# Autodesk Inventor assembly: EFS Mark I
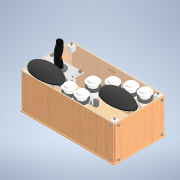
[picture p0: Inventor's stored thumbnail of the model, 180x180]
Saved by Autodesk Inventor 2022 (Build 260153000, 153)
## iProperties
Category: Gaming
Company: El Camino College
Created: 2023-03-29
Part Number: EFS Mark I
Document SubType Name: Assembly
Designer: Edgar Tejada
Project: Ergonomic Fight Stick
Mass: 952.379 g
Surface Area: 5483.02 cm^2
Volume: 844.231 cm^3
Density: 1.1281 g/cm^3
Author: Edgar Tejada
Title: Ergonomic Fight Stick
Keywords: Gaming Arcade Mame Ergonomic
## Documents named in this file (15)
- G:\Documents\Inventor HW\Ergonomic Fight Stick\Ergonomic_Fight_Stick.iam
- G:\Documents\Inventor HW\Ergonomic Fight Stick\Base_Plate.ipt
- G:\Documents\Inventor HW\Ergonomic Fight Stick\Vertical_Plate.ipt
- G:\Documents\Inventor HW\Ergonomic Fight Stick\Horizontal_Plate.ipt
- G:\Documents\Inventor HW\Ergonomic Fight Stick\Corner_M3_Mounts.ipt
- G:\Documents\Inventor HW\Ergonomic Fight Stick\AS 1420 - 1973 - M3 x 6.ipt
- G:\Documents\Inventor HW\Ergonomic Fight Stick\Top_Plate.ipt
- G:\Documents\Inventor HW\Ergonomic Fight Stick\Pushbutton - BG.iam
- G:\Documents\Inventor HW\Ergonomic Fight Stick\Sanwa JLF-TP-8YT 16Gate.iam
- G:\Documents\Inventor HW\Ergonomic Fight Stick\Makey_Makey_Circuit_Board.ipt
- C:\Users\brev\Documents\Inventor\Content Center Files\R2022\en-US\AS 1420\AS 1420 - 1973 - M3 x 10.ipt
- C:\Users\brev\Documents\Inventor\Content Center Files\R2022\en-US\BS 4183(1)\BS 4183 - M3(1).ipt
- G:\Documents\Inventor HW\Ergonomic Fight Stick\Nagasuye_Ergonomic_Controller_New_Grip.ipt
- G:\Documents\Inventor HW\Ergonomic Fight Stick\Silicone_Wrist_Support.ipt
- C:\Users\brev\Documents\Inventor\Content Center Files\R2022\en-US\SS-ISO 7093\ISO 7093 - 3 - 140 HV(2).ipt
## Components (67 placed, 14 different names)
1. Base_Plate:1 — Mate:1, Mate:2, Mate:3, Mate:4, Tangent:1, Tangent:2, Mate:5, Mate:6, Mate:7, Mate:8, Tangent:3, Tangent:4, Mate:9, Mate:10, Mate:11, Mate:12, Insert:3, Insert:6, Insert:8, Insert:9, Angle:4, Insert:32, Insert:33, Insert:34, Angle:8, Insert:35, Angle:10, Flush:1
2. Vertical_Plate:1 — Mate:1, Mate:3, Tangent:1, Insert:1, Insert:5, Angle:1, Insert:21, Insert:22
3. Vertical_Plate:2 — Mate:2, Mate:4, Tangent:2, Insert:12, Insert:13, Angle:3, Insert:19, Insert:25, Angle:5
4. Horizontal_Plate:3 — Mate:5, Mate:8, Tangent:4, Insert:7, Insert:11, Angle:2, Insert:23, Insert:24
5. Horizontal_Plate:4 — Mate:6, Mate:7, Tangent:3, Insert:10, Insert:17, Insert:18, Angle:6, Angle:9
6. AS 1420 - Metric M3 x 6:1 — Insert:1, Insert:2
7. AS 1420 - Metric M3 x 6:3 — Insert:4
8. AS 1420 - Metric M3 x 6:6 — Insert:11
9. AS 1420 - Metric M3 x 6:8 — Insert:13
10. AS 1420 - Metric M3 x 6:9 — Insert:7
11. AS 1420 - Metric M3 x 6:10 — Insert:10
12. AS 1420 - Metric M3 x 6:11 — Insert:12
13. AS 1420 - Metric M3 x 6:12 — Insert:5
14. AS 1420 - Metric M3 x 6:13 — Insert:17
15. AS 1420 - Metric M3 x 6:14 — Insert:18
16. AS 1420 - Metric M3 x 6:15 — Insert:19
17. AS 1420 - Metric M3 x 6:16 — Insert:25
18. AS 1420 - Metric M3 x 6:17 — Insert:21
19. AS 1420 - Metric M3 x 6:18 — Insert:22
20. AS 1420 - Metric M3 x 6:19 — Insert:24
21. AS 1420 - Metric M3 x 6:20 — Insert:23
22. Top_Plate:1 — Angle:4, Angle:5, Angle:6, Insert:26, Insert:27, Insert:28, Insert:29, Insert:30, Mate:13, Insert:31, Angle:7, Angle:10, Flush:1, Mate:15, Mate:16, Insert:39, Insert:40, Insert:41, Insert:42, Insert:43, Insert:44, Insert:45, Insert:46, Angle:11, Angle:12, Angle:14, Mate:19, Mate:20
23. Pushbutton - BG:1 [sub-assembly] — Insert:30
24. Pushbutton - BG:2 [sub-assembly] — Insert:29
25. Pushbutton - BG:3 [sub-assembly] — Mate:13
26. Pushbutton - BG:4 [sub-assembly] — Insert:28
27. Pushbutton - BG:5 [sub-assembly] — Insert:27
28. Pushbutton - BG:6 [sub-assembly] — Insert:26
29. Sanwa JLF-TP-8YT 16Gate:1 [sub-assembly] — Insert:31, Angle:7, Insert:51
30. AS 1420 - Metric M3 x 10:1 — Insert:32
31. AS 1420 - Metric M3 x 10:3 — Insert:34
32. AS 1420 - Metric M3 x 10:2 — Insert:33
33. Makey_Makey_Circuit_Board:1 — Angle:8, Insert:35, Angle:9, Insert:36, Insert:37, Insert:38
34. BS 4183 - Metric M3:1 — Insert:36
35. BS 4183 - Metric M3:2 — Insert:38
36. BS 4183 - Metric M3:3 — Insert:37
37. AS 1420 - Metric M3 x 6:5 — Insert:6, Insert:14
38. AS 1420 - Metric M3 x 6:7 — Insert:9, Insert:15
39. AS 1420 - Metric M3 x 6:4 — Insert:8, Insert:16
40. AS 1420 - Metric M3 x 6:2 — Insert:3
41. AS 1420 - Metric M3 x 6:21 — Insert:39, Insert:48, Insert:52
42. AS 1420 - Metric M3 x 6:22 — Insert:41, Insert:49, Insert:54
43. AS 1420 - Metric M3 x 6:23 — Insert:43
44. AS 1420 - Metric M3 x 6:24 — Insert:40, Insert:50, Insert:53
45. AS 1420 - Metric M3 x 6:25 — Insert:46
46. AS 1420 - Metric M3 x 6:26 — Insert:44
47. AS 1420 - Metric M3 x 6:27 — Insert:42, Insert:47, Insert:55
48. AS 1420 - Metric M3 x 6:28 — Insert:45
49. BS 4183 - Metric M3:4 — Insert:47
50. BS 4183 - Metric M3:5 — Insert:48
51. BS 4183 - Metric M3:6 — Insert:50
52. BS 4183 - Metric M3:7 — Insert:49
53. Nagasuye_Ergonomic_Controller_New_Grip:1 — Insert:51
54. Silicone_Wrist_Support:1 — Angle:11, Angle:13, Mate:19
55. Silicone_Wrist_Support:2 — Angle:12, Angle:13, Angle:14, Mate:20
56. SS ISO 7093 3 - 140 HV:1 — Insert:55
57. SS ISO 7093 3 - 140 HV:2 — Insert:54
58. SS ISO 7093 3 - 140 HV:3 — Insert:52
59. SS ISO 7093 3 - 140 HV:4 — Insert:53
60. Corner_M3_Mounts:4 — Mate:9, Insert:16, Angle:3
61. Corner_M3_Mounts:3 — Mate:12, Insert:2, Insert:4
62. Corner_M3_Mounts:1 — Mate:11, Insert:15, Angle:2
63. Corner_M3_Mounts:2 — Mate:10, Insert:14, Angle:1
64. Corner_M3_Mounts:5
65. Corner_M3_Mounts:6
66. Corner_M3_Mounts:7
67. Corner_M3_Mounts:8 — Mate:15, Mate:16
## Component patterns: (2 elements, first: Corner_M3_Mounts:4 + Corner_M3_Mounts:3 + Corner_M3_Mounts:1 + Corner_M3_Mounts:2)
## Relationships (90: Insert 54, Mate 17, Angle 14, Tangent 4, Flush 1)
- Mate:1: Base_Plate:1 ↔ Vertical_Plate:1
- Mate:2: Base_Plate:1 ↔ Vertical_Plate:2
- Mate:3: Base_Plate:1 ↔ Vertical_Plate:1
- Mate:4: Base_Plate:1 ↔ Vertical_Plate:2
- Tangent:1: Base_Plate:1 ↔ Vertical_Plate:1
- Tangent:2: Base_Plate:1 ↔ Vertical_Plate:2
- Mate:5: Base_Plate:1 ↔ Horizontal_Plate:3
- Mate:6: Base_Plate:1 ↔ Horizontal_Plate:4
- Mate:7: Base_Plate:1 ↔ Horizontal_Plate:4
- Mate:8: Base_Plate:1 ↔ Horizontal_Plate:3
- Tangent:3: Base_Plate:1 ↔ Horizontal_Plate:4
- Tangent:4: Base_Plate:1 ↔ Horizontal_Plate:3
- Mate:9: Base_Plate:1 ↔ Corner_M3_Mounts:4
- Mate:10: Base_Plate:1 ↔ Corner_M3_Mounts:2
- Mate:11: Base_Plate:1 ↔ Corner_M3_Mounts:1
- Mate:12: Base_Plate:1 ↔ Corner_M3_Mounts:3
- Insert:1: Vertical_Plate:1 ↔ AS 1420 - Metric M3 x 6:1
- Insert:2 (-2 mm): AS 1420 - Metric M3 x 6:1 ↔ Corner_M3_Mounts:3
- Insert:3 (-3 mm): Base_Plate:1 ↔ AS 1420 - Metric M3 x 6:2
- Insert:4 (-3 mm): AS 1420 - Metric M3 x 6:3 ↔ Corner_M3_Mounts:3
- Insert:5: Vertical_Plate:1 ↔ AS 1420 - Metric M3 x 6:12
- Insert:6: Base_Plate:1 ↔ AS 1420 - Metric M3 x 6:5
- Insert:7: Horizontal_Plate:3 ↔ AS 1420 - Metric M3 x 6:9
- Insert:8: Base_Plate:1 ↔ AS 1420 - Metric M3 x 6:4
- Insert:9: Base_Plate:1 ↔ AS 1420 - Metric M3 x 6:7
- Insert:10: Horizontal_Plate:4 ↔ AS 1420 - Metric M3 x 6:10
- Insert:11: Horizontal_Plate:3 ↔ AS 1420 - Metric M3 x 6:6
- Insert:12: Vertical_Plate:2 ↔ AS 1420 - Metric M3 x 6:11
- Insert:13: Vertical_Plate:2 ↔ AS 1420 - Metric M3 x 6:8
- Insert:14 (-2 mm): AS 1420 - Metric M3 x 6:5 ↔ Corner_M3_Mounts:2
- Angle:1 (0 deg): Vertical_Plate:1 ↔ Corner_M3_Mounts:2
- Insert:15 (-2 mm): AS 1420 - Metric M3 x 6:7 ↔ Corner_M3_Mounts:1
- Angle:2 (0 deg): Horizontal_Plate:3 ↔ Corner_M3_Mounts:1
- Insert:16 (-2 mm): AS 1420 - Metric M3 x 6:4 ↔ Corner_M3_Mounts:4
- Angle:3 (0 deg): Vertical_Plate:2 ↔ Corner_M3_Mounts:4
- Insert:17: Horizontal_Plate:4 ↔ AS 1420 - Metric M3 x 6:13
- Insert:18: Horizontal_Plate:4 ↔ AS 1420 - Metric M3 x 6:14
- Insert:19: Vertical_Plate:2 ↔ AS 1420 - Metric M3 x 6:15
- Insert:21: Vertical_Plate:1 ↔ AS 1420 - Metric M3 x 6:17
- Insert:22: Vertical_Plate:1 ↔ AS 1420 - Metric M3 x 6:18
- Insert:23: Horizontal_Plate:3 ↔ AS 1420 - Metric M3 x 6:20
- Insert:24: Horizontal_Plate:3 ↔ AS 1420 - Metric M3 x 6:19
- Insert:25: Vertical_Plate:2 ↔ AS 1420 - Metric M3 x 6:16
- Angle:4 (0 deg): Base_Plate:1 ↔ Top_Plate:1
- Angle:5 (0 deg): Vertical_Plate:2 ↔ Top_Plate:1
- Angle:6 (0 deg): Horizontal_Plate:4 ↔ Top_Plate:1
- Insert:26 (-3.5 mm): Top_Plate:1 ↔ Pushbutton - BG:6
- Insert:27 (-3.5 mm): Top_Plate:1 ↔ Pushbutton - BG:5
- Insert:28: Top_Plate:1 ↔ Pushbutton - BG:4
- Insert:29: Top_Plate:1 ↔ Pushbutton - BG:2
- Insert:30: Top_Plate:1 ↔ Pushbutton - BG:1
- Mate:13: Top_Plate:1 ↔ Pushbutton - BG:3
- Insert:31: Top_Plate:1 ↔ Sanwa JLF-TP-8YT 16Gate:1
- Angle:7 (0 deg): Top_Plate:1 ↔ Sanwa JLF-TP-8YT 16Gate:1
- Insert:32: Base_Plate:1 ↔ AS 1420 - Metric M3 x 10:1
- Insert:33: Base_Plate:1 ↔ AS 1420 - Metric M3 x 10:2
- Insert:34: Base_Plate:1 ↔ AS 1420 - Metric M3 x 10:3
- Angle:8 (0 deg): Base_Plate:1 ↔ Makey_Makey_Circuit_Board:1
- Insert:35 (2 mm): Base_Plate:1 ↔ Makey_Makey_Circuit_Board:1
- Angle:9 (0 deg): Horizontal_Plate:4 ↔ Makey_Makey_Circuit_Board:1
- Insert:36: Makey_Makey_Circuit_Board:1 ↔ BS 4183 - Metric M3:1
- Insert:37: Makey_Makey_Circuit_Board:1 ↔ BS 4183 - Metric M3:3
- Insert:38: Makey_Makey_Circuit_Board:1 ↔ BS 4183 - Metric M3:2
- Angle:10 (0 deg): Base_Plate:1 ↔ Top_Plate:1
- Flush:1: Base_Plate:1 ↔ Top_Plate:1
- Mate:15: Top_Plate:1 ↔ Corner_M3_Mounts:8
- Mate:16: Top_Plate:1 ↔ Corner_M3_Mounts:8
- Insert:39 (-0.8 mm): Top_Plate:1 ↔ AS 1420 - Metric M3 x 6:21
- Insert:40 (-0.8 mm): Top_Plate:1 ↔ AS 1420 - Metric M3 x 6:24
- Insert:41 (-0.8 mm): Top_Plate:1 ↔ AS 1420 - Metric M3 x 6:22
- Insert:42 (-0.8 mm): Top_Plate:1 ↔ AS 1420 - Metric M3 x 6:27
- Insert:43: Top_Plate:1 ↔ AS 1420 - Metric M3 x 6:23
- Insert:44: Top_Plate:1 ↔ AS 1420 - Metric M3 x 6:26
- Insert:45: Top_Plate:1 ↔ AS 1420 - Metric M3 x 6:28
- Insert:46: Top_Plate:1 ↔ AS 1420 - Metric M3 x 6:25
- Insert:47 (-2 mm): AS 1420 - Metric M3 x 6:27 ↔ BS 4183 - Metric M3:4
- Insert:48 (-2 mm): AS 1420 - Metric M3 x 6:21 ↔ BS 4183 - Metric M3:5
- Insert:49 (-2 mm): AS 1420 - Metric M3 x 6:22 ↔ BS 4183 - Metric M3:7
- Insert:50 (-2 mm): AS 1420 - Metric M3 x 6:24 ↔ BS 4183 - Metric M3:6
- Insert:51: Sanwa JLF-TP-8YT 16Gate:1 ↔ Nagasuye_Ergonomic_Controller_New_Grip:1
- Angle:11 (180 deg): Top_Plate:1 ↔ Silicone_Wrist_Support:1
- Angle:12 (180 deg): Top_Plate:1 ↔ Silicone_Wrist_Support:2
- Angle:13 (0 deg): Silicone_Wrist_Support:1 ↔ Silicone_Wrist_Support:2
- Angle:14 (0 deg): Top_Plate:1 ↔ Silicone_Wrist_Support:2
- Mate:19: Top_Plate:1 ↔ Silicone_Wrist_Support:1
- Mate:20: Top_Plate:1 ↔ Silicone_Wrist_Support:2
- Insert:52: AS 1420 - Metric M3 x 6:21 ↔ SS ISO 7093 3 - 140 HV:3
- Insert:53: AS 1420 - Metric M3 x 6:24 ↔ SS ISO 7093 3 - 140 HV:4
- Insert:54: AS 1420 - Metric M3 x 6:22 ↔ SS ISO 7093 3 - 140 HV:2
- Insert:55: AS 1420 - Metric M3 x 6:27 ↔ SS ISO 7093 3 - 140 HV:1
